# Autodesk Inventor assembly: main_sumec_assembly
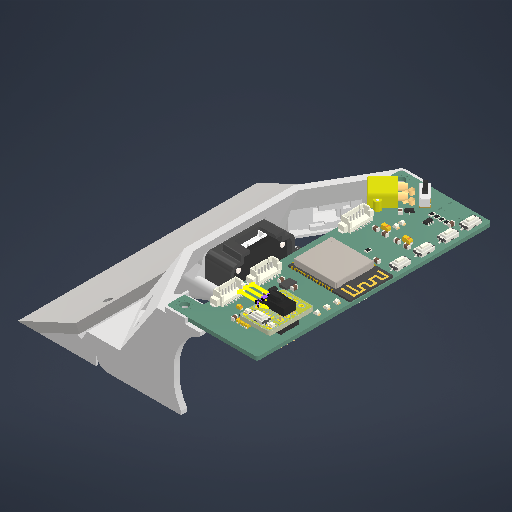
[picture p0: Inventor's stored thumbnail of the model, 512x512]
Saved by Autodesk Inventor 2025 (Build 290162000, 162)
## iProperties
Created: 2025-03-18
Part Number: main_sumec_assembly
Document SubType Name: Assembly
Designer: Simak
Author: Simak
## Documents named in this file (8)
- C:\_desktop\GitHub\Sumec-MiniSumo\-3D-\main_sumec_assembly.iam
- C:\_desktop\GitHub\Sumec-MiniSumo\-3D-\machined\lowerRamp.ipt
- C:\_desktop\GitHub\Sumec-MiniSumo\-3D-\screws\screws\M3_kuzel_torx\torx_socket_countersunk_flat_head_M3x08.ipt
- C:\_desktop\GitHub\Sumec-MiniSumo\-3D-\3D_printed\body-front.ipt
- C:\_desktop\GitHub\Sumec-MiniSumo\-3D-\electronics\pololu-digital-distance-sensor-irs17a.ipt
- C:\_desktop\GitHub\Sumec-MiniSumo\-3D-\electronics\AssemBeneWake TF-LUNA.ipt
- C:\_desktop\GitHub\Sumec-MiniSumo\-3D-\3D_printed\body-main.ipt
- C:\_desktop\GitHub\Sumec-MiniSumo\-3D-\electronics\PCBs\main board\SUMEC_MK_V .iam
## Components (9 placed, 7 different names)
1. lowerRamp:1 — Vložit:1, Vložit:2, Vložit:3, Proti sobě:1, Stejný směr:1, Stejný směr:2
2. torx_socket_countersunk_flat_head_M3x08:1 — Vložit:3
3. torx_socket_countersunk_flat_head_M3x08:2 — Vložit:1
4. torx_socket_countersunk_flat_head_M3x08:3 — Vložit:2
5. body-front:1 — Proti sobě:1, Stejný směr:1, Stejný směr:2, Stejný směr:3, Vložit:4, Vložit:5, Proti sobě:2, Stejný směr:4, Stejný směr:5, Vložit:6, Vložit:7, Stejný směr:6
6. pololu-digital-distance-sensor-irs17a:1 — Stejný směr:3, Vložit:4
7. AssemBeneWake TF-LUNA:1 — Vložit:5, Proti sobě:2
8. body-main:1 — Stejný směr:4, Stejný směr:5, Vložit:6
9. SUMEC_MK_V :1 [sub-assembly] — Vložit:7, Stejný směr:6
## Relationships (15: Insert 7, Flush 6, Mate 2)
- Vložit:1 [Insert] (0.5 mm): lowerRamp:1 ↔ torx_socket_countersunk_flat_head_M3x08:2
- Vložit:2 [Insert] (0.5 mm): lowerRamp:1 ↔ torx_socket_countersunk_flat_head_M3x08:3
- Vložit:3 [Insert] (0.5 mm): lowerRamp:1 ↔ torx_socket_countersunk_flat_head_M3x08:1
- Proti sobě:1 [Mate]: lowerRamp:1 ↔ body-front:1
- Stejný směr:1 [Flush]: lowerRamp:1 ↔ body-front:1
- Stejný směr:2 [Flush]: lowerRamp:1 ↔ body-front:1
- Stejný směr:3 [Flush]: body-front:1 ↔ pololu-digital-distance-sensor-irs17a:1
- Vložit:4 [Insert]: body-front:1 ↔ pololu-digital-distance-sensor-irs17a:1
- Vložit:5 [Insert]: body-front:1 ↔ AssemBeneWake TF-LUNA:1
- Proti sobě:2 [Mate]: body-front:1 ↔ AssemBeneWake TF-LUNA:1
- Stejný směr:4 [Flush]: body-front:1 ↔ body-main:1
- Stejný směr:5 [Flush]: body-front:1 ↔ body-main:1
- Vložit:6 [Insert]: body-front:1 ↔ body-main:1
- Vložit:7 [Insert]: body-front:1 ↔ SUMEC_MK_V :1
- Stejný směr:6 [Flush]: body-front:1 ↔ SUMEC_MK_V :1
